# Autodesk Inventor assembly: Corpo_Interno
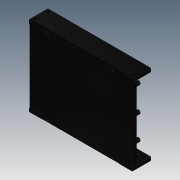
[picture p0: Inventor's stored thumbnail of the model, 180x180]
Saved by Autodesk Inventor 2020 (Build 240168000, 168)
## iProperties
Created: 2021-06-24
Part Number: Corpo_Interno
Document SubType Name: Assembly
Designer: JCarlos
Author: JCarlos
## Documents named in this file (4)
- C:\Users\candu\Google Drive\Doutorado_UTFPR\Projeto_1_SpotMicro\Projeto_3D\Robo_Montado_v3\3Dfiles_Q-Robot\Corpo_Interno_v3.iam
- C:\Users\candu\Google Drive\Doutorado_UTFPR\Projeto_1_SpotMicro\Projeto_3D\Robo_Montado_v3\3Dfiles_Q-Robot\Lateral.ipt
- C:\Users\candu\Google Drive\Doutorado_UTFPR\Projeto_1_SpotMicro\Projeto_3D\Robo_Montado_v3\3Dfiles_Q-Robot\Lateral_LadoUSB.ipt
- C:\Users\candu\Google Drive\Doutorado_UTFPR\Projeto_1_SpotMicro\Projeto_3D\Robo_Montado_v3\3Dfiles_Q-Robot\Base_Componentes_Arduino_v3.ipt
## Components (3 placed, 3 different names)
1. Base_Componentes_Arduino_v3:1 — Coincidência:1, Coincidência:3, Coincidência:15, Coincidência:18, Alinhamento:1, Coincidência:19, Coincidência:20
2. Lateral:2 — Coincidência:1, Coincidência:3, Coincidência:15
3. Lateral_LadoUSB:1 — Coincidência:18, Alinhamento:1, Coincidência:19
## Relationships (7: Mate 6, Flush 1)
- Coincidência:1 [Mate]: Base_Componentes_Arduino_v3:1 ↔ Lateral:2
- Coincidência:3 [Mate]: Base_Componentes_Arduino_v3:1 ↔ Lateral:2
- Coincidência:15 [Mate]: Base_Componentes_Arduino_v3:1 ↔ Lateral:2
- Coincidência:18 [Mate]: Base_Componentes_Arduino_v3:1 ↔ Lateral_LadoUSB:1
- Alinhamento:1 [Flush]: Base_Componentes_Arduino_v3:1 ↔ Lateral_LadoUSB:1
- Coincidência:19 [Mate]: Base_Componentes_Arduino_v3:1 ↔ Lateral_LadoUSB:1
- Coincidência:20 [Mate]: Base_Componentes_Arduino_v3:1
